# Autodesk Inventor assembly: RaisingCamJig
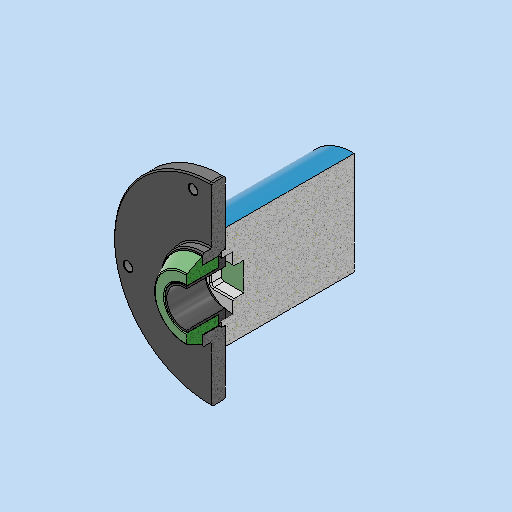
[picture p0: Inventor's stored thumbnail of the model, 512x512]
Saved by Autodesk Inventor 2025 (Build 290162000, 162)
## iProperties
Created: 2025-02-20
Part Number: RaisingCamJig
Document SubType Name: Assembly
Designer: kuzmin
Author: kuzmin
## Documents named in this file (5)
- C:\Users\queez\Dropbox\Drawings\PIHTI\Jobin-Yvon\RaisingCamJig.iam
- C:\Users\queez\Dropbox\Drawings\PIHTI\Jobin-Yvon\RisingCam-IMX571.ipt
- C:\Users\queez\Dropbox\Drawings\PIHTI\Jobin-Yvon\Jobin-Yvon-mounting-plate-RaisingCam.ipt
- C:\Users\queez\Dropbox\Drawings\PIHTI\Jobin-Yvon\M42-nose-peace.ipt
- C:\Users\queez\Dropbox\Drawings\PIHTI\Jobin-Yvon\TouptekAdapterCylinder.ipt
## Components (4 placed, 4 different names)
1. RisingCam-IMX571:1 — Mate:1, Flush:1, Rigid:1
2. Jobin-Yvon-mounting-plate-RaisingCam:1 — Mate:1, Flush:1
3. M42-nose-peace:1 — Rigid:1, Rigid:2
4. TouptekAdapterCylinder:1 — Rigid:2
## Relationships (4: WeldJoint 2, Mate 1, Flush 1)
- Mate:1: RisingCam-IMX571:1 ↔ Jobin-Yvon-mounting-plate-RaisingCam:1
- Flush:1 (25 mm): RisingCam-IMX571:1 ↔ Jobin-Yvon-mounting-plate-RaisingCam:1
- Rigid:1 [WeldJoint]: RisingCam-IMX571:1 ↔ M42-nose-peace:1
- Rigid:2 [WeldJoint]: M42-nose-peace:1 ↔ TouptekAdapterCylinder:1
